# Autodesk Inventor assembly: Assembly1
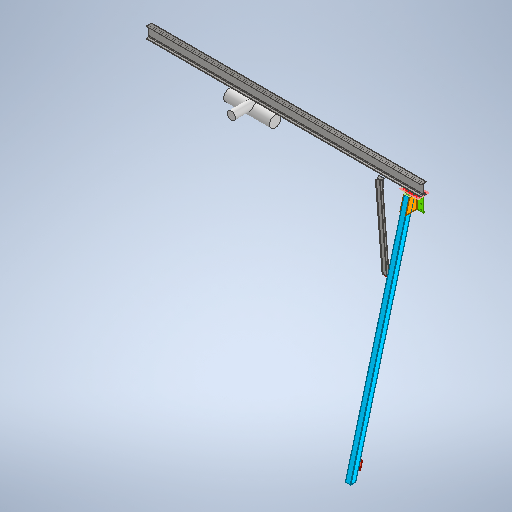
[picture p0: Inventor's stored thumbnail of the model, 512x512]
Saved by Autodesk Inventor 2025 (Build 290162010, 162A)
## iProperties
Created: 2024-06-11
Part Number: Assembly1
Document SubType Name: Assembly
Designer: admin
Author: admin
## Documents named in this file (9)
- C:\Users\admin\YandexDisk-badmisterfox\домашниий пк\Inventor\Workshop\оборудование\Кран козловой 2\Assembly1.iam
- C:\Users\admin\YandexDisk-badmisterfox\домашниий пк\Inventor\Workshop\оборудование\Двутавр 240x36 - 6000.ipt
- C:\Users\admin\YandexDisk-badmisterfox\домашниий пк\Inventor\Workshop\оборудование\Кран козловой 2\WRS 000,000 кран козловой 6х4.ipt
- C:\Users\admin\YandexDisk-badmisterfox\домашниий пк\Inventor\Workshop\оборудование\Кран козловой 2\Тельфер Таль электрическая.ipt
- C:\Users\admin\YandexDisk-badmisterfox\домашниий пк\Inventor\Workshop\оборудование\Кран козловой 2\Ухо на швеллер пямое.ipt
- C:\Users\admin\YandexDisk-badmisterfox\домашниий пк\Inventor\Workshop\оборудование\Кран козловой 2\Assembly2 стойка.iam
- C:\Users\admin\YandexDisk-badmisterfox\домашниий пк\Inventor\Workshop\оборудование\Кран козловой 2\Ухо на стойку_CPY_CPY.ipt
- C:\Users\admin\YandexDisk-badmisterfox\домашниий пк\Inventor\Workshop\оборудование\Кран козловой 2\JIS G 3192 - 100 x 50 x 5 - 1500 - 0,00936(4).ipt
- C:\Users\admin\YandexDisk-badmisterfox\домашниий пк\Inventor\Workshop\оборудование\Кран козловой 2\Ухо на стойку_CPY.ipt
## Components (9 placed, 8 different names)
1. Двутавр 240x36 - 6000:1 — Flush:1, Mate:1, Flush:2, Flush:4, Mate:15, Flush:17
2. WRS 000,000 кран козловой 6х4:1 — Mate:2, Mate:3, Flush:3
3. Тельфер Таль электрическая:1 — Flush:4, Mate:4
4. Ухо на швеллер пямое:1 — Mate:15, Flush:17, Flush:18
5. Assembly2 стойка:1 [sub-assembly] — Rotational:1, Mate:18
6. Ухо на стойку_CPY_CPY:1 — Flush:24, Flush:25, Mate:16, Rotational:1, Mate:18
7. JIS G 3192 - 100 x 50 x 5 - 1500 - 0,00936(4):1 — Flush:24, Flush:25, Mate:16, Flush:26, Flush:27, Mate:17
8. Ухо на стойку_CPY_CPY:2 — Flush:26, Flush:27, Mate:17, Rotational:2, Mate:19
9. Ухо на стойку_CPY:1 — Rotational:2, Mate:19
## Relationships (24: Flush 12, Mate 9, RevoluteJoint 2, WeldJoint 1)
- Flush:1 (4850 mm): Двутавр 240x36 - 6000:1
- Mate:1: Двутавр 240x36 - 6000:1
- Flush:2: Двутавр 240x36 - 6000:1
- Mate:2: WRS 000,000 кран козловой 6х4:1
- Mate:3: WRS 000,000 кран козловой 6х4:1
- Flush:3: WRS 000,000 кран козловой 6х4:1
- Flush:4: Двутавр 240x36 - 6000:1 ↔ Тельфер Таль электрическая:1
- Mate:4: Тельфер Таль электрическая:1
- [Flush]: Assembly2 стойка:1
- Mate:15: Двутавр 240x36 - 6000:1 ↔ Ухо на швеллер пямое:1
- Flush:17: Двутавр 240x36 - 6000:1 ↔ Ухо на швеллер пямое:1
- Flush:18: Ухо на швеллер пямое:1
- [Flush]: Assembly2 стойка:1
- [WeldJoint]: Ухо на швеллер пямое:1 ↔ Assembly2 стойка:1
- Flush:24: Ухо на стойку_CPY_CPY:1 ↔ JIS G 3192 - 100 x 50 x 5 - 1500 - 0,00936(4):1
- Flush:25: Ухо на стойку_CPY_CPY:1 ↔ JIS G 3192 - 100 x 50 x 5 - 1500 - 0,00936(4):1
- Mate:16: Ухо на стойку_CPY_CPY:1 ↔ JIS G 3192 - 100 x 50 x 5 - 1500 - 0,00936(4):1
- Flush:26: JIS G 3192 - 100 x 50 x 5 - 1500 - 0,00936(4):1 ↔ Ухо на стойку_CPY_CPY:2
- Flush:27: JIS G 3192 - 100 x 50 x 5 - 1500 - 0,00936(4):1 ↔ Ухо на стойку_CPY_CPY:2
- Mate:17: JIS G 3192 - 100 x 50 x 5 - 1500 - 0,00936(4):1 ↔ Ухо на стойку_CPY_CPY:2
- Rotational:1 [RevoluteJoint]: Assembly2 стойка:1 ↔ Ухо на стойку_CPY_CPY:1
- Mate:18: Assembly2 стойка:1 ↔ Ухо на стойку_CPY_CPY:1
- Rotational:2 [RevoluteJoint]: Ухо на стойку_CPY_CPY:2 ↔ Ухо на стойку_CPY:1
- Mate:19: Ухо на стойку_CPY_CPY:2 ↔ Ухо на стойку_CPY:1
